# Autodesk Inventor assembly: Z Endstop
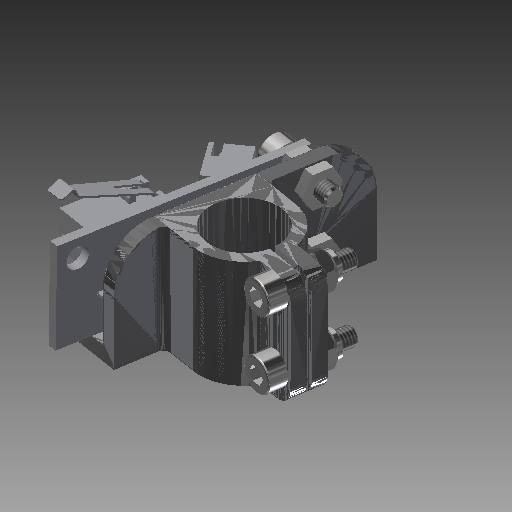
[picture p0: Inventor's stored thumbnail of the model, 512x512]
Saved by Autodesk Inventor 2018 (Build 220112000, 112)
## iProperties
Created: 2016-08-22
Part Number: Z Endstop
Document SubType Name: Assembly
Designer: User
Author: User
## Documents named in this file (7)
- C:\Users\Dan\OneDrive\SL-Inventor\The Beast v1.2 PackandGo\Workspaces\Workspace\Z Endstop.iam
- C:\Users\Dan\OneDrive\SL-Inventor\The Beast v1.2 PackandGo\Workspaces\Workspace\Z Endstop Holder.ipt
- C:\Users\Dan\OneDrive\SL-Inventor\The Beast v1.2 PackandGo\Workspaces\Workspace\en-US\ANSI B18.3.1M(6)\ANSI B18.3.1M - M3x0.5 x 12(1).ipt
- C:\Users\Dan\OneDrive\SL-Inventor\The Beast v1.2 PackandGo\Workspaces\Workspace\en-US\ANSI B18.16.3M(2)\ANSI B18.16.3M - Property Class 5 and 10 - Metric M3 x 0.5 Metal Type.ipt
- C:\Users\Dan\OneDrive\SL-Inventor\The Beast v1.2 PackandGo\Workspaces\Workspace\Capteur fin de course.ipt
- C:\Users\Dan\OneDrive\SL-Inventor\The Beast v1.2 PackandGo\Workspaces\Workspace\en-US\CSN EN 24 036\CSN EN 24 036 - M3.ipt
- C:\Users\Dan\OneDrive\SL-Inventor\The Beast v1.2 PackandGo\Workspaces\Workspace\en-US\ANSI B18.3.1M(6)\ANSI B18.3.1M - M3x0.5 x 10(1).ipt
## Components (12 placed, 6 different names)
1. Z Endstop Holder:1 — Mate:11, Mate:13
2. Forged Socket Head Cap Screw - Metric M3x0.5 x 12:1
3. Forged Socket Head Cap Screw - Metric M3x0.5 x 12:2
4. Prevailing Torque Type Hex Nut - Steel Metric Property Class 5 and 10 - Metric M3 x 0.5 Metal Type:1
5. Prevailing Torque Type Hex Nut - Steel Metric Property Class 5 and 10 - Metric M3 x 0.5 Metal Type:2
6. Capteur fin de course:1
7. Forged Socket Head Cap Screw - Metric M3x0.5 x 10:1 — Mate:10
8. Forged Socket Head Cap Screw - Metric M3x0.5 x 10:2 — Mate:12
9. CSN EN 24036 M3:1
10. CSN EN 24036 M3:2
11. CSN EN 24036 M3:3 — Mate:10, Mate:11
12. CSN EN 24036 M3:4 — Mate:12, Mate:13
## Relationships (17: Mate 13, Insert 4)
- [Insert]: Z Endstop Holder:1 ↔ Forged Socket Head Cap Screw - Metric M3x0.5 x 12:1
- [Insert]: Z Endstop Holder:1 ↔ Forged Socket Head Cap Screw - Metric M3x0.5 x 12:2
- [Mate]: Forged Socket Head Cap Screw - Metric M3x0.5 x 12:1 ↔ Prevailing Torque Type Hex Nut - Steel Metric Property Class 5 and 10 - Metric M3 x 0.5 Metal Type:1
- [Mate]: Z Endstop Holder:1 ↔ Prevailing Torque Type Hex Nut - Steel Metric Property Class 5 and 10 - Metric M3 x 0.5 Metal Type:1
- [Mate]: Forged Socket Head Cap Screw - Metric M3x0.5 x 12:2 ↔ Prevailing Torque Type Hex Nut - Steel Metric Property Class 5 and 10 - Metric M3 x 0.5 Metal Type:2
- [Mate]: Z Endstop Holder:1 ↔ Prevailing Torque Type Hex Nut - Steel Metric Property Class 5 and 10 - Metric M3 x 0.5 Metal Type:2
- [Insert]: Capteur fin de course:1 ↔ Forged Socket Head Cap Screw - Metric M3x0.5 x 10:1
- [Insert]: Capteur fin de course:1 ↔ Forged Socket Head Cap Screw - Metric M3x0.5 x 10:2
- [Mate]: Forged Socket Head Cap Screw - Metric M3x0.5 x 10:2 ↔ CSN EN 24036 M3:1
- [Mate]: Capteur fin de course:1 ↔ CSN EN 24036 M3:1
- [Mate]: Forged Socket Head Cap Screw - Metric M3x0.5 x 10:1 ↔ CSN EN 24036 M3:2
- [Mate]: Capteur fin de course:1 ↔ CSN EN 24036 M3:2
- [Mate]: Z Endstop Holder:1 ↔ CSN EN 24036 M3:1
- Mate:10: Forged Socket Head Cap Screw - Metric M3x0.5 x 10:1 ↔ CSN EN 24036 M3:3
- Mate:11: Z Endstop Holder:1 ↔ CSN EN 24036 M3:3
- Mate:12: Forged Socket Head Cap Screw - Metric M3x0.5 x 10:2 ↔ CSN EN 24036 M3:4
- Mate:13: Z Endstop Holder:1 ↔ CSN EN 24036 M3:4
